# Autodesk Inventor assembly: section_upper
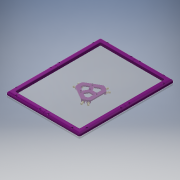
[picture p0: Inventor's stored thumbnail of the model, 180x180]
Saved by Autodesk Inventor 2017 (Build 210142000, 142)
## iProperties
Part Number: section_upper
Material: Ogólny
Document SubType Name: Assembly
Designer: Speed King
Mass: 932.858 g
Surface Area: 4038.55 cm^2
Volume: 672.087 cm^3
Density: 1.388 g/cm^3
Author: Speed King
## Documents named in this file (7)
- F:\Workspace\Inventor\Ti\CAD\model\section_upper.iam
- F:\Workspace\Inventor\Ti\CAD\model\plate_upper.ipt
- F:\Workspace\Inventor\Ti\CAD\model\frame_lower.ipt
- F:\Workspace\Inventor\Ti\CAD\model\resistive_panel_12.1.ipt
- F:\Workspace\Inventor\Ti\CAD\model\frame_upper.ipt
- F:\Workspace\Inventor\Ti\CAD\model\joint_ball_upper.ipt
- F:\Workspace\Inventor\Ti\CAD\model\frame_3d_asm.iam
## Components (11 placed, 6 different names)
1. plate_upper:1 — Zestawiający:1, Zestawiający:2, Kąt:1, Zestawiający:3, Zestawiający:4, Kąt:2, Zestawiający:5, Zestawiający:6, Kąt:3, Zestawiający:7, Zestawiający:8, Kąt:4, Zestawiający:9, Zestawiający:10, Kąt:5, Zestawiający:11, Zestawiający:12, Kąt:6, Zestawiający:13, Zestawiający:14, Zestawiający:15, Równoległy:1, Równoległy:2
2. joint_ball_upper:1 — Zestawiający:3, Zestawiający:4, Kąt:2
3. joint_ball_upper:2 — Zestawiający:5, Zestawiający:6, Kąt:3
4. joint_ball_upper:3 — Zestawiający:7, Zestawiający:8, Kąt:4
5. joint_ball_upper:4 — Zestawiający:11, Zestawiający:12, Kąt:6, Zestawiający:22
6. joint_ball_upper:5 — Zestawiający:9, Zestawiający:10, Kąt:5
7. joint_ball_upper:6 — Zestawiający:1, Zestawiający:2, Kąt:1
8. frame_upper:1 — Zestawiający:19, Zestawiający:20, Zestawiający:21
9. frame_lower:1 — Zestawiający:13, Zestawiający:14, Zestawiający:15, Zestawiający:16, Zestawiający:17, Zestawiający:18, Zestawiający:19, Zestawiający:20
10. resistive_panel_12.1:1 — Zestawiający:16, Zestawiający:17, Zestawiający:18, Zestawiający:21, Zestawiający:23, Równoległy:3, Równoległy:4
11. frame_3d_asm:1 [sub-assembly] — Zestawiający:23, Równoległy:3, Równoległy:4
## Relationships (33: Mate 23, Angle 6, Flush 4)
- Zestawiający:1 [Mate]: plate_upper:1 ↔ joint_ball_upper:6
- Zestawiający:2 [Mate]: plate_upper:1 ↔ joint_ball_upper:6
- Kąt:1 [Angle] (0 deg): plate_upper:1 ↔ joint_ball_upper:6
- Zestawiający:3 [Mate]: plate_upper:1 ↔ joint_ball_upper:1
- Zestawiający:4 [Mate]: plate_upper:1 ↔ joint_ball_upper:1
- Kąt:2 [Angle] (0 deg): plate_upper:1 ↔ joint_ball_upper:1
- Zestawiający:5 [Mate]: plate_upper:1 ↔ joint_ball_upper:2
- Zestawiający:6 [Mate]: plate_upper:1 ↔ joint_ball_upper:2
- Kąt:3 [Angle] (0 deg): plate_upper:1 ↔ joint_ball_upper:2
- Zestawiający:7 [Mate]: plate_upper:1 ↔ joint_ball_upper:3
- Zestawiający:8 [Mate]: plate_upper:1 ↔ joint_ball_upper:3
- Kąt:4 [Angle] (0 deg): plate_upper:1 ↔ joint_ball_upper:3
- Zestawiający:9 [Mate]: plate_upper:1 ↔ joint_ball_upper:5
- Zestawiający:10 [Mate]: plate_upper:1 ↔ joint_ball_upper:5
- Kąt:5 [Angle] (0 deg): plate_upper:1 ↔ joint_ball_upper:5
- Zestawiający:11 [Mate]: plate_upper:1 ↔ joint_ball_upper:4
- Zestawiający:12 [Mate]: plate_upper:1 ↔ joint_ball_upper:4
- Kąt:6 [Angle] (0 deg): plate_upper:1 ↔ joint_ball_upper:4
- Zestawiający:13 [Mate]: plate_upper:1 ↔ frame_lower:1
- Zestawiający:14 [Mate]: plate_upper:1 ↔ frame_lower:1
- Zestawiający:15 [Mate]: plate_upper:1 ↔ frame_lower:1
- Zestawiający:16 [Mate]: frame_lower:1 ↔ resistive_panel_12.1:1
- Zestawiający:17 [Mate]: frame_lower:1 ↔ resistive_panel_12.1:1
- Zestawiający:18 [Mate]: frame_lower:1 ↔ resistive_panel_12.1:1
- Zestawiający:19 [Mate]: frame_upper:1 ↔ frame_lower:1
- Zestawiający:20 [Mate]: frame_upper:1 ↔ frame_lower:1
- Zestawiający:21 [Mate]: frame_upper:1 ↔ resistive_panel_12.1:1
- Równoległy:1 [Flush]: plate_upper:1
- Równoległy:2 [Flush]: plate_upper:1
- Zestawiający:22 [Mate]: joint_ball_upper:4
- Zestawiający:23 [Mate]: resistive_panel_12.1:1 ↔ frame_3d_asm:1
- Równoległy:3 [Flush]: resistive_panel_12.1:1 ↔ frame_3d_asm:1
- Równoległy:4 [Flush] (0.5 mm): resistive_panel_12.1:1 ↔ frame_3d_asm:1
